# Autodesk Inventor assembly: Assembly
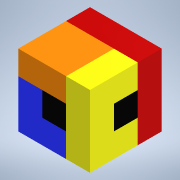
[picture p0: Inventor's stored thumbnail of the model, 180x180]
Saved by Autodesk Inventor 2020 (Build 240168000, 168)
## iProperties
Created: 2019-12-20
Part Number: Assembly
Document SubType Name: Assembly
Designer: Corey
Author: Corey
## Documents named in this file (6)
- C:\Users\Corey\Documents\IED_2019\Puzzle Cube\Assembly.iam
- C:\Users\Corey\Documents\IED_2019\Puzzle Cube\Corner.ipt
- C:\Users\Corey\Documents\IED_2019\Puzzle Cube\Square with Lobe.ipt
- C:\Users\Corey\Documents\IED_2019\Puzzle Cube\Stair.ipt
- C:\Users\Corey\Documents\IED_2019\Puzzle Cube\U with Lobe.ipt
- C:\Users\Corey\Documents\IED_2019\Puzzle Cube\U.ipt
## Components (5 placed, 5 different names)
1. Corner:1 — Flush:3, Flush:4, Mate:5, Mate:6
2. Square with Lobe:1 — Flush:1, Mate:1, Mate:2, Mate:3, Mate:5, Flush:5
3. Stair:1 — Flush:2, Mate:3, Mate:4, Mate:7
4. U with Lobe:1 — Flush:1, Mate:1, Mate:2, Flush:2, Mate:4, Flush:3, Flush:4
5. U:1 — Mate:6, Flush:5, Mate:7
## Relationships (12: Mate 7, Flush 5)
- Flush:1: Square with Lobe:1 ↔ U with Lobe:1
- Mate:1: Square with Lobe:1 ↔ U with Lobe:1
- Mate:2: Square with Lobe:1 ↔ U with Lobe:1
- Flush:2: Stair:1 ↔ U with Lobe:1
- Mate:3: Square with Lobe:1 ↔ Stair:1
- Mate:4: Stair:1 ↔ U with Lobe:1
- Flush:3: Corner:1 ↔ U with Lobe:1
- Flush:4: Corner:1 ↔ U with Lobe:1
- Mate:5: Corner:1 ↔ Square with Lobe:1
- Mate:6: Corner:1 ↔ U:1
- Flush:5: Square with Lobe:1 ↔ U:1
- Mate:7: Stair:1 ↔ U:1
